# Autodesk Inventor assembly: ABC-2020-4
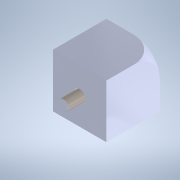
[picture p0: Inventor's stored thumbnail of the model, 180x180]
Saved by Autodesk Inventor 2021.1 (Build 251245010, 245A)
## iProperties
Created: 2020-11-06
Part Number: ABC-2020-4
Document SubType Name: Assembly
Designer: gisen
Sending System: SOLIDWORKS 2016-2016095
MC: AMD64
MC_MODEL: Intel64 Family 6 Model 45 Stepping 7, GenuineIntel
OS: Windows_NT
FRU: Parasolid Version 28.0, build 209,  1-25-2016
FORMAT: text
GUISE: transmit
KEY: ABC-2020-4
FILE: ABC-2020-4.x_t
DATE: Thu Aug 18 09:44:38 2016
Author: gisen
## Documents named in this file (4)
- C:\Users\gisen\GitProjects\CAD-Data\GeneralComponentsTemplate\Fittings\BasicFrameCubeBracket.iam
- C:\Users\gisen\GitProjects\CAD-Data\GeneralComponentsTemplate\Fittings\BasicFrameCubeBracket\ABC-2020-4_BR.ipt
- C:\Users\gisen\GitProjects\CAD-Data\GeneralComponentsTemplate\Fittings\BasicFrameCubeBracket\ABC-2020-4_cover.ipt
- C:\Users\gisen\GitProjects\CAD-Data\GeneralComponentsTemplate\Fittings\BasicFrameCubeBracket\CS-04.ipt
## Components (5 placed, 3 different names)
1. ABC-2020-4_BR — メイト:1, メイト:2, メイト:3, メイト:4, メイト:5, メイト:6, フラッシュ:1, フラッシュ:2, フラッシュ:3
2. ABC-2020-4_cover — フラッシュ:1, フラッシュ:2, フラッシュ:3
3. CS-04 — メイト:3, メイト:4
4. CS-04:1 — メイト:1, メイト:2
5. CS-04:2 — メイト:5, メイト:6
## Relationships (9: Mate 6, Flush 3)
- メイト:1 [Mate]: ABC-2020-4_BR ↔ CS-04:1
- メイト:2 [Mate]: ABC-2020-4_BR ↔ CS-04:1
- メイト:3 [Mate]: ABC-2020-4_BR ↔ CS-04
- メイト:4 [Mate]: ABC-2020-4_BR ↔ CS-04
- メイト:5 [Mate]: ABC-2020-4_BR ↔ CS-04:2
- メイト:6 [Mate]: ABC-2020-4_BR ↔ CS-04:2
- フラッシュ:1 [Flush]: ABC-2020-4_BR ↔ ABC-2020-4_cover
- フラッシュ:2 [Flush]: ABC-2020-4_BR ↔ ABC-2020-4_cover
- フラッシュ:3 [Flush]: ABC-2020-4_BR ↔ ABC-2020-4_cover
